# Autodesk Inventor assembly: Cyl_Lens_OnPost
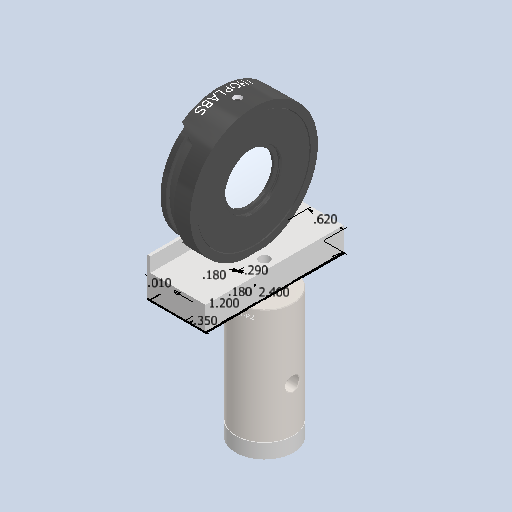
[picture p0: Inventor's stored thumbnail of the model, 512x512]
Saved by Autodesk Inventor 2024.2 (Build 282272000, 272)
## iProperties
Created: 2024-01-29
Part Number: Cyl_Lens_OnPost
Document SubType Name: Assembly
Designer: monolithic
Author: monolithic
## Documents named in this file (5)
- C:\Users\monolithic\Documents\GitHub\CAD\Monolith\John\ASLM_SampleScanning_Baseplate\Assembly\Components\SubAssemblies\Cyl_Lens_OnPost.iam
- C:\Users\monolithic\Documents\GitHub\CAD\Monolith\John\ASLM_SampleScanning_Baseplate\Assembly\Components\SubAssemblies\PLS-P2.ipt
- C:\Users\monolithic\Documents\GitHub\CAD\Monolith\John\ASLM_SampleScanning_Baseplate\Assembly\Components\SubAssemblies\PolarisPost_HeightAdjustment_0p25in_smallholesfrom0p79to0p81.ipt
- C:\Users\monolithic\Documents\GitHub\CAD\Monolith\John\ASLM_SampleScanning_Baseplate\Assembly\Components\SubAssemblies\RSP1toPolarisPinAdapter.ipt
- C:\Users\monolithic\Documents\GitHub\CAD\Monolith\John\ASLM_SampleScanning_Baseplate\Assembly\Components\SubAssemblies\Cyl_Lens_Holder.iam
## Components (4 placed, 4 different names)
1. PLS-P2:1 — Mate:1, Mate:2, Mate:3, Mate:4, Mate:5
2. PolarisPost_HeightAdjustment_0p25in_smallholesfrom0p79to0p81:1 — Mate:1, Mate:2
3. RSP1toPolarisPinAdapter:1 — Mate:3, Mate:4, Mate:5, Mate:6, Angle:1
4. Cyl_Lens_Holder:1 [sub-assembly] — Mate:6, Angle:1
## Relationships (7: Mate 6, Angle 1)
- Mate:1: PLS-P2:1 ↔ PolarisPost_HeightAdjustment_0p25in_smallholesfrom0p79to0p81:1
- Mate:2: PLS-P2:1 ↔ PolarisPost_HeightAdjustment_0p25in_smallholesfrom0p79to0p81:1
- Mate:3: PLS-P2:1 ↔ RSP1toPolarisPinAdapter:1
- Mate:4: PLS-P2:1 ↔ RSP1toPolarisPinAdapter:1
- Mate:5: PLS-P2:1 ↔ RSP1toPolarisPinAdapter:1
- Mate:6: RSP1toPolarisPinAdapter:1 ↔ Cyl_Lens_Holder:1
- Angle:1 (180 deg): RSP1toPolarisPinAdapter:1 ↔ Cyl_Lens_Holder:1
